# Autodesk Inventor assembly: 200-60-DIFFERENTIAL-BAR-01
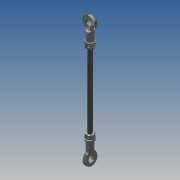
[picture p0: Inventor's stored thumbnail of the model, 180x180]
Saved by Autodesk Inventor 2018.2 (Build 222227000, 227)
## iProperties
Manager: feesmrt
Company: FRANCOR
Part Number: 200-60-DIFFERENTIAL-BAR-01
Project: Rescue Robot
Cost Center: -
Material: Generisch
Document SubType Name: Assembly
Designer: feesmrt
Engineer: feesmrt
Authority: feesmrt
Description: Differential Verbinder ASM
Stock Number: 200-60-DIFFERENTIAL-BAR-01
Subject: Rescue Robot
Author: feesmrt
Revision Number: 1
Title: Differential Verbinder ASM
## Documents named in this file (4)
- D:\Programmierung\FRANC0R\CAD\02-Rocker-Bogie-Robot\200-ROCKER-BOGIE\200-60-DIFFERENTIAL\200-60-DIFFERENTIAL-BAR-01.iam
- D:\Programmierung\FRANC0R\CAD\02-Rocker-Bogie-Robot\200-ROCKER-BOGIE\200-60-DIFFERENTIAL\200-60-DIFFERENTIAL-BAR-05.ipt
- D:\Programmierung\FRANC0R\CAD\02-Rocker-Bogie-Robot\900-COMPONENTS\900-41-NUTS\900-41-NUTS-ISO4035-M8.ipt
- D:\Programmierung\FRANC0R\CAD\02-Rocker-Bogie-Robot\900-COMPONENTS\900-70-ANGLE-JOINTS\900-70-ANGLE-JOINT-DIN648-M8-1.ipt
## Components (7 placed, 3 different names)
1. 200-60-DIFFERENTIAL-BAR-05:1 — Passend:1, Passend:2, Passend:9, Passend:10, Passend:11, Passend:12
2. 900-70-ANGLE-JOINT-DIN648-M8-1:1 — Passend:1, Passend:3, Passend:5, Passend:7, Passend:10
3. 900-70-ANGLE-JOINT-DIN648-M8-1:2 — Passend:2, Passend:4, Passend:6, Passend:9, Passend:15
4. 900-41-NUTS-ISO4035-M8:1 — Passend:3, Passend:5, Passend:14
5. 900-41-NUTS-ISO4035-M8:2 — Passend:4, Passend:6, Passend:13
6. 900-41-NUTS-ISO4035-M8:3 — Passend:12, Passend:13
7. 900-41-NUTS-ISO4035-M8:4 — Passend:11, Passend:14
## Relationships (14: Mate 14)
- Passend:1 [Mate]: 200-60-DIFFERENTIAL-BAR-05:1 ↔ 900-70-ANGLE-JOINT-DIN648-M8-1:1
- Passend:2 [Mate]: 200-60-DIFFERENTIAL-BAR-05:1 ↔ 900-70-ANGLE-JOINT-DIN648-M8-1:2
- Passend:3 [Mate]: 900-70-ANGLE-JOINT-DIN648-M8-1:1 ↔ 900-41-NUTS-ISO4035-M8:1
- Passend:4 [Mate]: 900-70-ANGLE-JOINT-DIN648-M8-1:2 ↔ 900-41-NUTS-ISO4035-M8:2
- Passend:5 [Mate]: 900-70-ANGLE-JOINT-DIN648-M8-1:1 ↔ 900-41-NUTS-ISO4035-M8:1
- Passend:6 [Mate]: 900-70-ANGLE-JOINT-DIN648-M8-1:2 ↔ 900-41-NUTS-ISO4035-M8:2
- Passend:7 [Mate]: 900-70-ANGLE-JOINT-DIN648-M8-1:1
- Passend:9 [Mate] (-13.5 mm): 200-60-DIFFERENTIAL-BAR-05:1 ↔ 900-70-ANGLE-JOINT-DIN648-M8-1:2
- Passend:10 [Mate] (-13.5 mm): 200-60-DIFFERENTIAL-BAR-05:1 ↔ 900-70-ANGLE-JOINT-DIN648-M8-1:1
- Passend:11 [Mate]: 200-60-DIFFERENTIAL-BAR-05:1 ↔ 900-41-NUTS-ISO4035-M8:4
- Passend:12 [Mate]: 200-60-DIFFERENTIAL-BAR-05:1 ↔ 900-41-NUTS-ISO4035-M8:3
- Passend:13 [Mate]: 900-41-NUTS-ISO4035-M8:2 ↔ 900-41-NUTS-ISO4035-M8:3
- Passend:14 [Mate]: 900-41-NUTS-ISO4035-M8:1 ↔ 900-41-NUTS-ISO4035-M8:4
- Passend:15 [Mate]: 900-70-ANGLE-JOINT-DIN648-M8-1:2
